# Autodesk Inventor assembly: Display
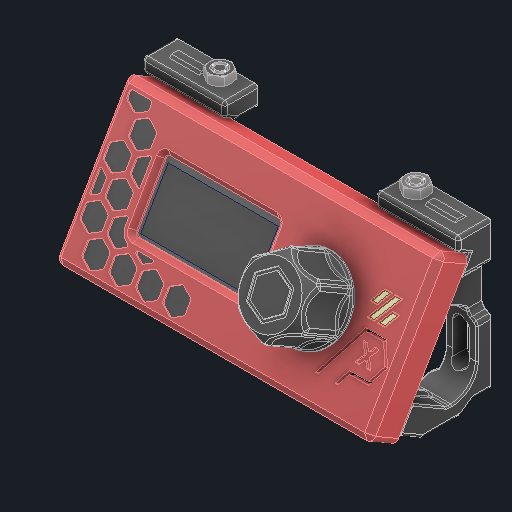
[picture p0: Inventor's stored thumbnail of the model, 512x512]
Saved by Autodesk Inventor 2025.1 (Build 291241020, 241B)
## iProperties
Created: 2025-05-09
Part Number: Display
Document SubType Name: Assembly
Designer: AdminForWorker
Title: Display
Author: AdminForWorker
## Documents named in this file (9)
- C:\Users\Joshua Eah\Documents\Voron 0.2\CAD\Master Assembly\Display.iam
- C:\Users\Joshua Eah\Documents\Voron 0.2\CAD\Master Assembly\V0 Display PCB.ipt
- C:\Users\Joshua Eah\Documents\Voron 0.2\CAD\Master Assembly\Hardware\M2x10 Self Tapper.ipt
- C:\Users\Joshua Eah\Documents\Voron 0.2\CAD\Master Assembly\Hardware\M3x6 BHCS.ipt
- C:\Users\Joshua Eah\Documents\Voron 0.2\CAD\Master Assembly\Hardware\M3 Hexnut.ipt
- C:\Users\Joshua Eah\Documents\Voron 0.2\CAD\Master Assembly\Display Diffuser.ipt
- C:\Users\Joshua Eah\Documents\Voron 0.2\CAD\Master Assembly\Display Faceplate.ipt
- C:\Users\Joshua Eah\Documents\Voron 0.2\CAD\Master Assembly\Encoder Knob.ipt
- C:\Users\Joshua Eah\Documents\Voron 0.2\CAD\Master Assembly\Display Mounts.ipt
## Components (13 placed, 8 different names)
1. Display Faceplate:1 — Mate:1, Mate:2, Mate:3, Insert:9, Insert:10, Mate:6, Mate:7, Angle:1
2. V0 Display PCB:1 — Insert:9, Insert:10, Mate:4, Mate:5
3. Display Mounts:1 — Mate:3
4. Display Diffuser:1 — Mate:6, Mate:7, Angle:1
5. Encoder Knob:1 — Mate:4, Mate:5
6. M2x10 Self Tapper:1
7. M2x10 Self Tapper:2 — Mate:2
8. M2x10 Self Tapper:3
9. M2x10 Self Tapper:4 — Mate:1
10. M3x6 BHCS:1 — Insert:5
11. M3x6 BHCS:2 — Insert:6
12. M3 Hexnut:1 — Insert:5
13. M3 Hexnut:2 — Insert:6
## Relationships (18: Insert 10, Mate 7, Angle 1)
- [Insert]: Display Mounts:1 ↔ M2x10 Self Tapper:1
- [Insert]: Display Mounts:1 ↔ M2x10 Self Tapper:4
- [Insert]: Display Mounts:1 ↔ M2x10 Self Tapper:2
- [Insert]: Display Mounts:1 ↔ M2x10 Self Tapper:3
- Insert:5: M3x6 BHCS:1 ↔ M3 Hexnut:1
- Insert:6: M3x6 BHCS:2 ↔ M3 Hexnut:2
- [Insert]: Display Mounts:1 ↔ M3x6 BHCS:1
- [Insert]: Display Mounts:1 ↔ M3x6 BHCS:2
- Mate:1: Display Faceplate:1 ↔ M2x10 Self Tapper:4
- Mate:2: Display Faceplate:1 ↔ M2x10 Self Tapper:2
- Mate:3: Display Faceplate:1 ↔ Display Mounts:1
- Insert:9: Display Faceplate:1 ↔ V0 Display PCB:1
- Insert:10: Display Faceplate:1 ↔ V0 Display PCB:1
- Mate:4: V0 Display PCB:1 ↔ Encoder Knob:1
- Mate:5: V0 Display PCB:1 ↔ Encoder Knob:1
- Mate:6: Display Faceplate:1 ↔ Display Diffuser:1
- Mate:7: Display Faceplate:1 ↔ Display Diffuser:1
- Angle:1 (0 deg): Display Faceplate:1 ↔ Display Diffuser:1
